# Autodesk Inventor assembly: ASTRAIOSAssembly
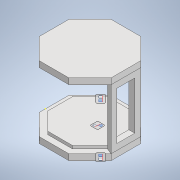
[picture p0: Inventor's stored thumbnail of the model, 180x180]
Saved by Autodesk Inventor 2020 (Build 240168000, 168)
## iProperties
Created: 2020-02-24
Part Number: ASTRAIOSAssembly
Document SubType Name: Assembly
Designer: WANG
Author: WANG
## Documents named in this file (4)
- C:\Users\ianwa\Documents\GitHub\ASTRAIOS\workspace\ASTRAIOSAssembly.iam
- C:\Users\ianwa\Documents\GitHub\ASTRAIOS\workspace\SatelliteTopFace.ipt
- C:\Users\ianwa\Documents\GitHub\ASTRAIOS\workspace\SatelliteBottomFace.ipt
- C:\Users\ianwa\Documents\GitHub\ASTRAIOS\workspace\SatelliteSideWall.ipt
## Components (3 placed, 3 different names)
1. SatelliteBottomFace:1 — Flush:1, Flush:2, Flush:3, Flush:4, Mate:1, Mate:3
2. SatelliteTopFace:2 — Flush:1, Flush:2, Flush:3, Flush:4, Mate:1, Mate:2, Mate:4
3. SatelliteSideWall:1 — Mate:2, Mate:3, Mate:4
## Relationships (8: Flush 4, Mate 4)
- Flush:1: SatelliteBottomFace:1 ↔ SatelliteTopFace:2
- Flush:2: SatelliteBottomFace:1 ↔ SatelliteTopFace:2
- Flush:3: SatelliteBottomFace:1 ↔ SatelliteTopFace:2
- Flush:4: SatelliteBottomFace:1 ↔ SatelliteTopFace:2
- Mate:1 (114.3 mm): SatelliteBottomFace:1 ↔ SatelliteTopFace:2
- Mate:2: SatelliteTopFace:2 ↔ SatelliteSideWall:1
- Mate:3: SatelliteBottomFace:1 ↔ SatelliteSideWall:1
- Mate:4: SatelliteTopFace:2 ↔ SatelliteSideWall:1
